# Autodesk Inventor assembly: Gearbox
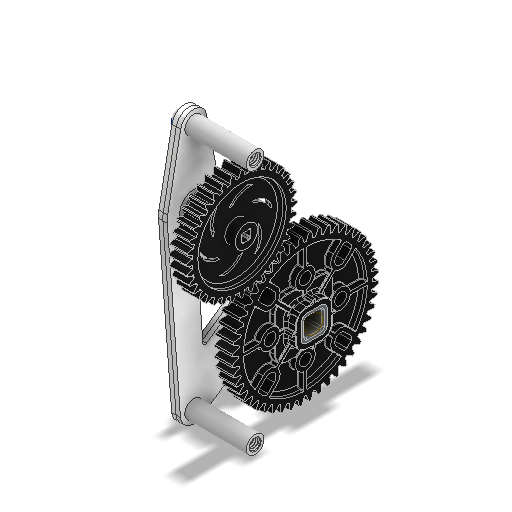
[picture p0: Inventor's stored thumbnail of the model, 512x512]
Saved by Autodesk Inventor 2025.2 (Build 292293000, 293)
## iProperties
Created: 2025-02-17
Part Number: Gearbox
Document SubType Name: Assembly
Designer: avere
Author: avere
## Documents named in this file (11)
- C:\Users\avere\VEX-CAD\V5-CAD\Conveyer\Gearbox.iam
- C:\Users\avere\VEX-CAD\ROBOPROS-CAD-Inventor\Motion\Insert Circle.ipt
- C:\Users\avere\VEX-CAD\V5-CAD\Conveyer\Custom Parts\Gearbox.ipt
- C:\Users\avere\VEX-CAD\ROBOPROS-CAD-Inventor\Structure\Nylon Standoff Rounded\Nylon Standoff .875.ipt
- C:\Users\avere\VEX-CAD\ROBOPROS-CAD-Inventor\Structure\Hardware\Screw Alu - Slotted\AScrew Slotted Threaded .250.ipt
- C:\Users\avere\VEX-CAD\ROBOPROS-CAD-Inventor\Structure\Hardware\Nut Alu.ipt
- C:\Users\avere\VEX-CAD\ROBOPROS-CAD-Inventor\Motion\Gears\LS 36T Gear.ipt
- C:\Users\avere\VEX-CAD\ROBOPROS-CAD-Inventor\Motion\Shaft LS\Shaft Collar ipts\Shaft Collar Set Screw.ipt
- C:\Users\avere\VEX-CAD\ROBOPROS-CAD-Inventor\Motion\Spacers\Washer Steel\SWasher .375 OD x .062500.ipt
- C:\Users\avere\VEX-CAD\ROBOPROS-CAD-Inventor\Motion\Spacers\Washer Steel.ipt
- C:\Users\avere\VEX-CAD\ROBOPROS-CAD-Inventor\Modified Parts\Equal Half Cut HS 48T Gear, No Insert.ipt
## Components (15 placed, 9 different names)
1. Insert Circle:1 — Mate:11
2. Gearbox:1 — Insert:2, Insert:3, Flush:1, Insert:6
3. Insert Circle:2 — Mate:8, Mate:10, Insert:8
4. Gearbox:2 — Insert:4, Insert:5, Insert:7
5. Nylon Standoff .875:1 — Insert:2
6. Nylon Standoff .875:2 — Insert:3, Mate:9
7. AScrew Slotted Threaded .250:1 — Insert:4
8. AScrew Slotted Threaded .250:2 — Insert:5
9. AScrew Slotted Threaded .250:3 — Insert:6
10. Nut Alu:1 — Insert:7
11. LS 36T Gear:1 — Insert:8, Insert:9, Flush:2
12. Shaft Collar Set Screw:1 — Insert:9, Insert:10
13. SWasher .375 OD x .062500:1 — Insert:10
14. Equal Half Cut HS 48T Gear, No Insert:1 — Mate:11, Flush:2, Insert:11
15. Shaft Collar Set Screw:2 — Insert:11
## Relationships (24: Mate 11, Insert 11, Flush 2)
- [Mate]: Insert Circle:1 ↔ Gearbox:1
- [Mate]: Insert Circle:1 ↔ Gearbox:1
- [Mate]: Insert Circle:1 ↔ Gearbox:1
- [Mate]: Gearbox:1 ↔ Insert Circle:2
- [Mate]: Gearbox:1 ↔ Insert Circle:2
- [Mate]: Gearbox:1 ↔ Insert Circle:2
- [Insert]: Gearbox:1 ↔ Gearbox:2
- [Mate]: Gearbox:1 ↔ Gearbox:2
- Insert:2: Gearbox:1 ↔ Nylon Standoff .875:1
- Insert:3: Gearbox:1 ↔ Nylon Standoff .875:2
- Flush:1: Gearbox:1
- Mate:8: Insert Circle:2
- Mate:9: Nylon Standoff .875:2
- Mate:10: Insert Circle:2
- Insert:4: Gearbox:2 ↔ AScrew Slotted Threaded .250:1
- Insert:5: Gearbox:2 ↔ AScrew Slotted Threaded .250:2
- Insert:6: Gearbox:1 ↔ AScrew Slotted Threaded .250:3
- Insert:7: Gearbox:2 ↔ Nut Alu:1
- Insert:8 (8.255 mm): Insert Circle:2 ↔ LS 36T Gear:1
- Insert:9: LS 36T Gear:1 ↔ Shaft Collar Set Screw:1
- Insert:10: Shaft Collar Set Screw:1 ↔ SWasher .375 OD x .062500:1
- Mate:11: Insert Circle:1 ↔ Equal Half Cut HS 48T Gear, No Insert:1
- Flush:2 (-1.5875 mm): LS 36T Gear:1 ↔ Equal Half Cut HS 48T Gear, No Insert:1
- Insert:11: Equal Half Cut HS 48T Gear, No Insert:1 ↔ Shaft Collar Set Screw:2
